# Autodesk Inventor assembly: Fixture_lin_mid_print
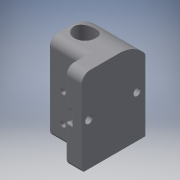
[picture p0: Inventor's stored thumbnail of the model, 180x180]
Saved by Autodesk Inventor 2019.3 (Build 233278000, 278)
## iProperties
Created: 2020-08-27
Part Number: Fixture_lin_mid_print
Material: Generisch
Document SubType Name: Assembly
Designer: Nicolas Frick
Author: Nicolas Frick
## Documents named in this file (2)
- C:\Users\Nicolas Frick\Sync\OneDrive\airhockeybot\mechanical_design\common_cad_parts\print_models\Fixture_lin_mid_print.iam
- C:\Users\Nicolas Frick\Sync\OneDrive\airhockeybot\mechanical_design\inventor\Fixture_linear_mid.ipt
## Components (1 placed, 1 different names)
1. Fixture_linear_mid:1 — Passend:1, Passend:2, Fluchtend:1
## Relationships (3: Mate 2, Flush 1)
- Passend:1 [Mate]: Fixture_linear_mid:1
- Passend:2 [Mate]: Fixture_linear_mid:1
- Fluchtend:1 [Flush]: Fixture_linear_mid:1
